# Autodesk Inventor assembly: Base
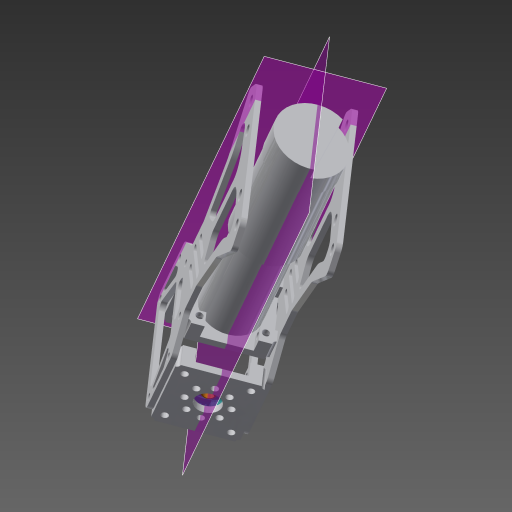
[picture p0: Inventor's stored thumbnail of the model, 512x512]
Saved by Autodesk Inventor 2023 (Build 270158000, 158)
## iProperties
Created: 2020-03-24
Part Number: Base
Document SubType Name: Assembly
Designer: valer
Mass: 4853.13 g
Surface Area: 3141.52 cm^2
Volume: 1403.99 cm^3
Density: 3.45667 g/cm^3
Author: valer
## Documents named in this file (8)
- C:\Users\Val\Desktop\drummingrobot\src\parts\export\Base.iam
- C:\Users\Val\Desktop\drummingrobot\src\parts\external\ShoulderServo.ipt
- C:\Users\Val\Desktop\drummingrobot\src\parts\external\ShoulderMiterGear.ipt
- C:\Users\Val\Desktop\drummingrobot\src\parts\external\ShoulderServoShaft.ipt
- C:\Users\Val\Desktop\drummingrobot\src\parts\external\ShoulderMotorMount.ipt
- C:\Users\Val\Desktop\drummingrobot\src\parts\external\PatternSpacer.ipt
- C:\Users\Val\Desktop\drummingrobot\src\parts\ShoulderBracket2.ipt
- C:\Users\Val\Desktop\drummingrobot\src\parts\external\Potentiometer\Potentiometer.iam
## Components (10 placed, 7 different names)
1. ShoulderServo:1 — Mate:301, Mate:367, Mate:368
2. ShoulderMiterGear:1 — Mate:303, Mate:369
3. ShoulderServoShaft:1 — Mate:301, Mate:303, Mate:316, Mate:367
4. ShoulderMotorMount:1 — Mate:316, Mate:326, Mate:365, Mate:366, Mate:368, Mate:369
5. ShoulderMotorMount:2 — Mate:321, Mate:323, Mate:324, Mate:325, Mate:328, Mate:364, Mate:370, Mate:371
6. PatternSpacer:1 — Mate:321, Mate:363, Mate:370, Mate:371, Flush:1
7. ShoulderBracket2:1 — Mate:323, Mate:324, Mate:325, Mate:365, Mate:366, Mate:373
8. ShoulderBracket2:2 — Mate:326, Mate:328, Mate:359, Mate:360, Mate:361, Mate:364, Angle:1
9. ShoulderMotorMount:3 — Mate:359, Mate:360, Mate:361, Mate:372, Mate:373, Mate:374, Angle:2
10. Potentiometer:1 [sub-assembly] — Mate:372, Mate:374, Angle:2
## Relationships (27: Mate 24, Angle 2, Flush 1)
- Mate:301: ShoulderServo:1 ↔ ShoulderServoShaft:1
- Mate:303: ShoulderMiterGear:1 ↔ ShoulderServoShaft:1
- Mate:316: ShoulderServoShaft:1 ↔ ShoulderMotorMount:1
- Mate:321: ShoulderMotorMount:2 ↔ PatternSpacer:1
- Mate:323: ShoulderMotorMount:2 ↔ ShoulderBracket2:1
- Mate:324: ShoulderMotorMount:2 ↔ ShoulderBracket2:1
- Mate:325: ShoulderMotorMount:2 ↔ ShoulderBracket2:1
- Mate:326: ShoulderMotorMount:1 ↔ ShoulderBracket2:2
- Mate:328: ShoulderMotorMount:2 ↔ ShoulderBracket2:2
- Mate:359: ShoulderBracket2:2 ↔ ShoulderMotorMount:3
- Mate:360: ShoulderBracket2:2 ↔ ShoulderMotorMount:3
- Mate:361: ShoulderBracket2:2 ↔ ShoulderMotorMount:3
- Mate:363: PatternSpacer:1
- Mate:364: ShoulderMotorMount:2 ↔ ShoulderBracket2:2
- Mate:365: ShoulderMotorMount:1 ↔ ShoulderBracket2:1
- Mate:366: ShoulderMotorMount:1 ↔ ShoulderBracket2:1
- Mate:367 (-4 mm): ShoulderServo:1 ↔ ShoulderServoShaft:1
- Mate:368: ShoulderServo:1 ↔ ShoulderMotorMount:1
- Mate:369 (1 mm): ShoulderMiterGear:1 ↔ ShoulderMotorMount:1
- Mate:370: ShoulderMotorMount:2 ↔ PatternSpacer:1
- Mate:371: ShoulderMotorMount:2 ↔ PatternSpacer:1
- Mate:372: ShoulderMotorMount:3 ↔ Potentiometer:1
- Mate:373: ShoulderBracket2:1 ↔ ShoulderMotorMount:3
- Flush:1: PatternSpacer:1
- Angle:1 (180 deg): ShoulderBracket2:2
- Mate:374: ShoulderMotorMount:3 ↔ Potentiometer:1
- Angle:2 (0 deg): ShoulderMotorMount:3 ↔ Potentiometer:1
